# Autodesk Inventor assembly: ensamble guante
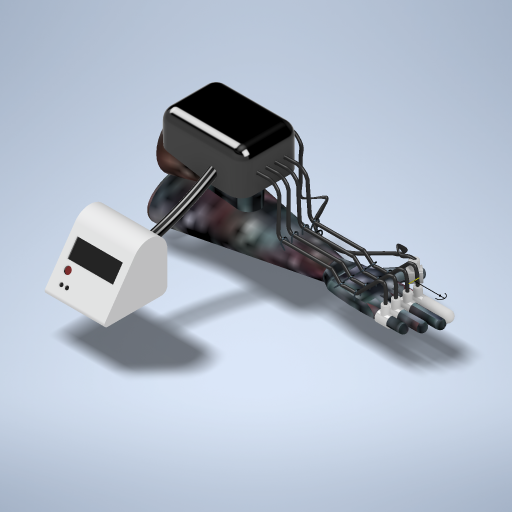
[picture p0: Inventor's stored thumbnail of the model, 512x512]
Saved by Autodesk Inventor 2023 (Build 270158000, 158)
## iProperties
Created: 2022-10-12
Part Number: ensamble guante
Document SubType Name: Assembly
Designer: Xiaba
Author: Xiaba
## Documents named in this file (13)
- C:\Users\Xiaba\Desktop\FUNBIO\Guante\ensamble guante.iam
- C:\Users\Xiaba\Desktop\FUNBIO\Guante\guante.ipt
- C:\Users\Xiaba\Desktop\FUNBIO\Guante\cajas de aire.ipt
- C:\Users\Xiaba\Desktop\FUNBIO\Guante\tubo.ipt
- C:\Users\Xiaba\Desktop\FUNBIO\Guante\cilindros de dedos.ipt
- C:\Users\Xiaba\Desktop\FUNBIO\Guante\cilindros de dedo gordo.ipt
- C:\Users\Xiaba\Desktop\FUNBIO\Guante\tubo chiquito.ipt
- C:\Users\Xiaba\Desktop\FUNBIO\Guante\caja del arduino.ipt
- C:\Users\Xiaba\Desktop\FUNBIO\Guante\soporte.ipt
- C:\Users\Xiaba\Desktop\FUNBIO\Guante\enrrollables.ipt
- C:\Users\Xiaba\Desktop\FUNBIO\Guante\ARDUINO.ipt
- C:\Users\Xiaba\Desktop\FUNBIO\Guante\cable de caja de arduino.ipt
- C:\Users\Xiaba\Desktop\FUNBIO\Guante\continuacion indice.ipt
## Components (33 placed, 12 different names)
1. guante:1 — Mate:10, Mate:12, Mate:13, Mate:14, Angle:1, Mate:18, Mate:19, Mate:20, Tangent:1, Tangent:2
2. tubo:1 — Mate:17, Mate:29, Mate:30, Mate:35, Mate:38, Mate:42, Mate:45, Mate:46, Mate:47
3. tubo:2 — Mate:15, Mate:32, Mate:36, Mate:40, Mate:44, Mate:49, Mate:52
4. tubo:3 — Mate:11, Mate:33, Mate:34, Mate:41, Mate:43, Mate:50, Mate:51
5. tubo:4 — Mate:16, Mate:31, Mate:37, Mate:39, Mate:48, Mate:53
6. cilindros de dedos:1 — Mate:10, Mate:11, Mate:54, Mate:55
7. cilindros de dedos:2 — Mate:12, Mate:15
8. cilindros de dedos:3 — Mate:13, Mate:16
9. cilindros de dedos:4 — Mate:14, Mate:17
10. cilindros de dedo gordo:1
11. tubo chiquito:1
12. caja del arduino:1
13. soporte:1 — Mate:29, Mate:30
14. soporte:2 — Mate:31
15. soporte:3 — Mate:32
16. soporte:4 — Mate:33
17. soporte:5 — Mate:37
18. soporte:6 — Mate:36
19. soporte:7 — Mate:35
20. soporte:8 — Mate:34
21. soporte:9 — Mate:38, Mate:42
22. soporte:10 — Mate:40
23. soporte:11 — Mate:41, Mate:43
24. soporte:12 — Mate:39
25. soporte:13
26. cajas de aire:3 — Mate:44, Mate:45
27. enrrollables:1 — Mate:46, Mate:47
28. enrrollables:2 — Mate:50, Mate:51
29. enrrollables:3 — Mate:49, Mate:52
30. enrrollables:4 — Mate:48, Mate:53
31. ARDUINO:1
32. cable de caja de arduino:1
33. continuacion indice:1 — Mate:54, Mate:55
## Relationships (44: Mate 38, Angle 3, Tangent 2, Flush 1)
- Mate:10: guante:1 ↔ cilindros de dedos:1
- Mate:11: tubo:3 ↔ cilindros de dedos:1
- Mate:12: guante:1 ↔ cilindros de dedos:2
- Mate:13: guante:1 ↔ cilindros de dedos:3
- Mate:14: guante:1 ↔ cilindros de dedos:4
- Mate:15: tubo:2 ↔ cilindros de dedos:2
- Mate:16: tubo:4 ↔ cilindros de dedos:3
- Mate:17: tubo:1 ↔ cilindros de dedos:4
- Angle:1 (0 deg): guante:1
- Mate:18: guante:1
- Mate:19: guante:1
- Angle:2 (180 deg)
- Mate:20: guante:1
- Tangent:1: guante:1
- Flush:2 (-1 mm)
- Angle:3 (0 deg)
- Tangent:2: guante:1
- Mate:29: tubo:1 ↔ soporte:1
- Mate:30: tubo:1 ↔ soporte:1
- Mate:31: tubo:4 ↔ soporte:2
- Mate:32: tubo:2 ↔ soporte:3
- Mate:33: tubo:3 ↔ soporte:4
- Mate:34: tubo:3 ↔ soporte:8
- Mate:35: tubo:1 ↔ soporte:7
- Mate:36: tubo:2 ↔ soporte:6
- Mate:37: tubo:4 ↔ soporte:5
- Mate:38: tubo:1 ↔ soporte:9
- Mate:39: tubo:4 ↔ soporte:12
- Mate:40: tubo:2 ↔ soporte:10
- Mate:41: tubo:3 ↔ soporte:11
- Mate:42: tubo:1 ↔ soporte:9
- Mate:43: tubo:3 ↔ soporte:11
- Mate:44: tubo:2 ↔ cajas de aire:3
- Mate:45: tubo:1 ↔ cajas de aire:3
- Mate:46: tubo:1 ↔ enrrollables:1
- Mate:47: tubo:1 ↔ enrrollables:1
- Mate:48: tubo:4 ↔ enrrollables:4
- Mate:49: tubo:2 ↔ enrrollables:3
- Mate:50: tubo:3 ↔ enrrollables:2
- Mate:51: tubo:3 ↔ enrrollables:2
- Mate:52: tubo:2 ↔ enrrollables:3
- Mate:53: tubo:4 ↔ enrrollables:4
- Mate:54: cilindros de dedos:1 ↔ continuacion indice:1
- Mate:55: cilindros de dedos:1 ↔ continuacion indice:1
